# Autodesk Inventor assembly: Pickup Arm Left
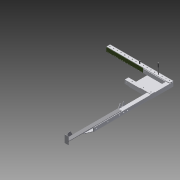
[picture p0: Inventor's stored thumbnail of the model, 180x180]
Saved by Autodesk Inventor 2015 (Build 190159000, 159)
## iProperties
Created: 2015-01-27
Part Number: Pickup Arm Left
Document SubType Name: Assembly
Designer: Admin
Author: Admin
## Documents named in this file (15)
- C:\Users\Jarod\Documents\Robotics\FRC\2015\CAD\Robot\Pickup Arms\Pickup Arm Left.iam
- C:\Users\Jarod\Documents\Robotics\FRC\2015\CAD\Robot\Pickup Arms\pickup arm 1x1.ipt
- C:\Users\Jarod\Documents\Robotics\FRC\2015\CAD\Robot\Pickup Arms\pickup arm plate.ipt
- C:\Users\Jarod\Documents\Robotics\FRC\2015\CAD\Robot\Pickup Arms\1x1 pickup arm support.ipt
- C:\Users\Jarod\Documents\Robotics\FRC\2015\CAD\Robot\Pickup Arms\rack.ipt
- C:\Users\Jarod\Documents\Robotics\FRC\2015\CAD\Robot\Pickup Arms\pickup arm gusset.ipt
- C:\Users\Jarod\Documents\Robotics\FRC\2015\CAD\Robot\Pickup Arms\spacer.ipt
- C:\Users\Jarod\Documents\Robotics\FRC\2015\CAD\Robot\Pickup Arms\1x1 pickup arm support rear.ipt
- C:\Users\Jarod\Documents\Robotics\FRC\2015\CAD\Robot\Pickup Arms\mechanical stop bolt.ipt
- C:\Users\Jarod\Documents\Robotics\FRC\2015\CAD\Robot\Pickup Arms\pickup arm tab.ipt
- C:\Users\Jarod\Documents\Robotics\FRC\2015\CAD\Robot\Pickup Arms\C-Channel.ipt
- C:\Users\Jarod\Documents\Robotics\FRC\2015\CAD\Robot\Pickup Arms\rubber grip.ipt
- C:\Users\Jarod\Documents\Robotics\FRC\2015\CAD\Robot\Pickup Arms\beam breaker bolt.ipt
- C:\Users\Jarod\Documents\Robotics\FRC\2015\CAD\Robot\Pickup Arms\front tab 2x2_MIR.ipt
- C:\Users\Jarod\Documents\Robotics\FRC\2015\CAD\Robot\Pickup Arms\1x1 angle arm extender.ipt
## Components (14 placed, 14 different names)
1. pickup arm 1x1:1 — Mate:1, Flush:1, Flush:2, Mate:2, Mate:12, Flush:7, Mate:13, Mate:15, Mate:16, Mate:18, Mate:22, Flush:11, Flush:13, Mate:27, Mate:33, Mate:34, Mate:35, Mate:40
2. pickup arm plate:1 — Mate:1, Flush:1, Flush:2, Mate:4, Flush:4, Mate:19, Mate:20
3. 1x1 pickup arm support:1 — Mate:2, Mate:4, Flush:4
4. 1x1 pickup arm support rear:1 — Mate:18, Mate:28, Mate:29
5. rack:1 — Mate:36, Mate:37, Flush:14
6. C-Channel:1 — Flush:13, Mate:26, Mate:27, Mate:28, Mate:29, Mate:36, Mate:37, Mate:38, Mate:39, Flush:14
7. pickup arm gusset:1 — Mate:12, Flush:7, Mate:13
8. spacer:1 — Mate:15, Mate:16, Mate:26
9. mechanical stop bolt:1 — Mate:19, Mate:20
10. beam breaker bolt:1 — Mate:38, Mate:39
11. front tab 2x2_MIR:1 — Mate:47, Mate:48, Flush:15
12. pickup arm tab:2 — Mate:22, Flush:11, Mate:40
13. rubber grip:1 — Mate:33, Mate:34, Mate:35
14. 1x1 angle arm extender:1 — Mate:47, Mate:48, Flush:15
## Relationships (36: Mate 28, Flush 8)
- Mate:1: pickup arm 1x1:1 ↔ pickup arm plate:1
- Flush:1: pickup arm 1x1:1 ↔ pickup arm plate:1
- Flush:2: pickup arm 1x1:1 ↔ pickup arm plate:1
- Mate:2: pickup arm 1x1:1 ↔ 1x1 pickup arm support:1
- Mate:4: pickup arm plate:1 ↔ 1x1 pickup arm support:1
- Flush:4: pickup arm plate:1 ↔ 1x1 pickup arm support:1
- Mate:12: pickup arm 1x1:1 ↔ pickup arm gusset:1
- Flush:7: pickup arm 1x1:1 ↔ pickup arm gusset:1
- Mate:13: pickup arm 1x1:1 ↔ pickup arm gusset:1
- Mate:15: pickup arm 1x1:1 ↔ spacer:1
- Mate:16: pickup arm 1x1:1 ↔ spacer:1
- Mate:18: pickup arm 1x1:1 ↔ 1x1 pickup arm support rear:1
- Mate:19: pickup arm plate:1 ↔ mechanical stop bolt:1
- Mate:20: pickup arm plate:1 ↔ mechanical stop bolt:1
- Mate:22: pickup arm 1x1:1 ↔ pickup arm tab:2
- Flush:11: pickup arm 1x1:1 ↔ pickup arm tab:2
- Flush:13: pickup arm 1x1:1 ↔ C-Channel:1
- Mate:26: C-Channel:1 ↔ spacer:1
- Mate:27: pickup arm 1x1:1 ↔ C-Channel:1
- Mate:28: 1x1 pickup arm support rear:1 ↔ C-Channel:1
- Mate:29 (3.175 mm): 1x1 pickup arm support rear:1 ↔ C-Channel:1
- Mate:33: pickup arm 1x1:1 ↔ rubber grip:1
- Mate:34: pickup arm 1x1:1 ↔ rubber grip:1
- Mate:35: pickup arm 1x1:1 ↔ rubber grip:1
- Mate:36: rack:1 ↔ C-Channel:1
- Mate:37 (3.175 mm): rack:1 ↔ C-Channel:1
- Mate:38: C-Channel:1 ↔ beam breaker bolt:1
- Mate:39: C-Channel:1 ↔ beam breaker bolt:1
- Mate:40: pickup arm 1x1:1 ↔ pickup arm tab:2
- Flush:14: rack:1 ↔ C-Channel:1
- [Mate]: pickup arm 1x1:1 ↔ 1x1 angle arm extender:1
- [Mate]: pickup arm 1x1:1 ↔ 1x1 angle arm extender:1
- [Mate]: pickup arm tab:2 ↔ 1x1 angle arm extender:1
- Mate:47: front tab 2x2_MIR:1 ↔ 1x1 angle arm extender:1
- Mate:48: front tab 2x2_MIR:1 ↔ 1x1 angle arm extender:1
- Flush:15: front tab 2x2_MIR:1 ↔ 1x1 angle arm extender:1
